# Autodesk Inventor assembly: ArmEncoderBoard
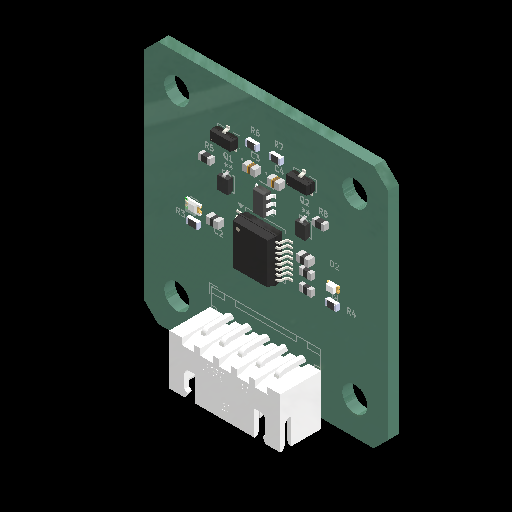
[picture p0: Inventor's stored thumbnail of the model, 512x512]
Saved by Autodesk Inventor 2025.2 (Build 292293000, 293)
## iProperties
Company: Kicad
Created: 2026-02-13
Part Number: ArmEncoderBoard
Description: KiCad electronic assembly
Document SubType Name: Assembly
Designer: valer
Authority: Unknown
Sending System: KiCad to STEP converter
Preprocessor: Open CASCADE STEP processor 7.8
Title: ArmEncoderBoardLatest.step
Author: Pcbnew
## Documents named in this file (18)
- C:\Users\valer\Desktop\str1ker\cad\external\ArmEncoder\ArmEncoderBoard.iam
- C:\Users\valer\Desktop\str1ker\cad\external\ArmEncoder\CC0603KRX7R9BB104.ipt
- C:\Users\valer\Desktop\str1ker\cad\external\ArmEncoder\CRCW0603100KFKEA.ipt
- C:\Users\valer\Desktop\str1ker\cad\external\ArmEncoder\CR0603-FX-4701ELF.ipt
- C:\Users\valer\Desktop\str1ker\cad\external\ArmEncoder\RC0603FR-0747KL.ipt
- C:\Users\valer\Desktop\str1ker\cad\external\ArmEncoder\150080BS75000.iam
- C:\Users\valer\Desktop\str1ker\cad\external\ArmEncoder\SOT-23.ipt
- C:\Users\valer\Desktop\str1ker\cad\external\ArmEncoder\SN74LVC2G17DBVR.iam
- C:\Users\valer\Desktop\str1ker\cad\external\ArmEncoder\SSOP-16_5.3x6.2mm_P0.65mm.ipt
- C:\Users\valer\Desktop\str1ker\cad\external\ArmEncoder\NCD0603R1.iam
- C:\Users\valer\Desktop\str1ker\cad\external\ArmEncoder\RC0603FR-07150RL.ipt
- C:\Users\valer\Desktop\str1ker\cad\external\ArmEncoder\RCG06031K00FKEA.ipt
- C:\Users\valer\Desktop\str1ker\cad\external\ArmEncoder\CC0603JRX7R7BB105.ipt
- C:\Users\valer\Desktop\str1ker\cad\external\ArmEncoder\BAT54WS-7-F.ipt
- C:\Users\valer\Desktop\str1ker\cad\external\ArmEncoder\ArmEncoderBoard_silkscreen.ipt
- C:\Users\valer\Desktop\str1ker\cad\external\ArmEncoder\ArmEncoderBoard_silkscreen_1.ipt
- C:\Users\valer\Desktop\str1ker\cad\external\ArmEncoder\ArmEncoderBoard_PCB.ipt
- C:\Users\valer\Desktop\str1ker\cad\external\ArmEncoder\WHITE JST XH 5 PIN CONNECTOR - P 2.54mm - ANGLED.ipt
## Components (24 placed, 24 different names)
1. 1
2. 2
3. 3
4. 4
5. 5
6. 12 [sub-assembly]
7. 13
8. 21 [sub-assembly]
9. 22
10. 28 [sub-assembly]
11. 30
12. 31
13. 32
14. 33
15. 34
16. 35
17. 36
18. 37
19. 38
20. 39
21. 40
22. 41
23. Board — Mate:1, Flush:1
24. WHITE JST XH 5 PIN CONNECTOR - P 2.54mm - ANGLED:1 — Mate:1, Flush:1
## Relationships (2: Mate 1, Flush 1)
- Mate:1: Board ↔ WHITE JST XH 5 PIN CONNECTOR - P 2.54mm - ANGLED:1
- Flush:1: Board ↔ WHITE JST XH 5 PIN CONNECTOR - P 2.54mm - ANGLED:1
